# Autodesk Inventor assembly: GarageAndBracket
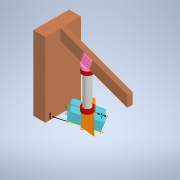
[picture p0: Inventor's stored thumbnail of the model, 180x180]
Saved by Autodesk Inventor 2022.2 (Build 262287000, 287)
## iProperties
Created: 2021-11-26
Part Number: GarageAndBracket
Document SubType Name: Assembly
Designer: robst
Author: robst
## Documents named in this file (7)
- C:\git\CAD-Development\robSteele\ShapeWays\GlobalMeteorNetwork\GarageAndBracket.iam
- C:\git\CAD-Development\robSteele\ShapeWays\GlobalMeteorNetwork\GarageSegment.ipt
- C:\git\CAD-Development\robSteele\ShapeWays\GlobalMeteorNetwork\pvcBracketUpperPortionV02.ipt
- C:\git\CAD-Development\robSteele\ShapeWays\GlobalMeteorNetwork\topAttachementForPvcPipe.ipt
- C:\git\CAD-Development\robSteele\ShapeWays\GlobalMeteorNetwork\2inchPvcForBracket.ipt
- C:\git\CAD-Development\robSteele\ShapeWays\GlobalMeteorNetwork\bracketForGarageLowerHalf.ipt
- C:\git\CAD-Development\robSteele\ShapeWays\GlobalMeteorNetwork\caseUpperPortion.ipt
## Components (7 placed, 6 different names)
1. GarageSegment:1 — Mate:1, Mate:2, Mate:3
2. pvcBracketUpperPortionV02:1 — Mate:1, Mate:2, Mate:3, Insert:1
3. 2inchPvcForBracket:1 — Mate:5, Mate:10, Insert:2
4. topAttachementForPvcPipe:1 — Mate:5, Mate:10, Insert:1
5. topAttachementForPvcPipe:2 — Insert:2, Mate:11
6. bracketForGarageLowerHalf:1 — Mate:11, Mate:12, Flush:1
7. caseUpperPortion:1 — Mate:12, Flush:1
## Relationships (10: Mate 7, Insert 2, Flush 1)
- Mate:1: GarageSegment:1 ↔ pvcBracketUpperPortionV02:1
- Mate:2: GarageSegment:1 ↔ pvcBracketUpperPortionV02:1
- Mate:3 (-254 mm): GarageSegment:1 ↔ pvcBracketUpperPortionV02:1
- Mate:5: 2inchPvcForBracket:1 ↔ topAttachementForPvcPipe:1
- Mate:10: 2inchPvcForBracket:1 ↔ topAttachementForPvcPipe:1
- Insert:1: pvcBracketUpperPortionV02:1 ↔ topAttachementForPvcPipe:1
- Insert:2: 2inchPvcForBracket:1 ↔ topAttachementForPvcPipe:2
- Mate:11: topAttachementForPvcPipe:2 ↔ bracketForGarageLowerHalf:1
- Mate:12: bracketForGarageLowerHalf:1 ↔ caseUpperPortion:1
- Flush:1: bracketForGarageLowerHalf:1 ↔ caseUpperPortion:1
